# Autodesk Inventor assembly: Gear
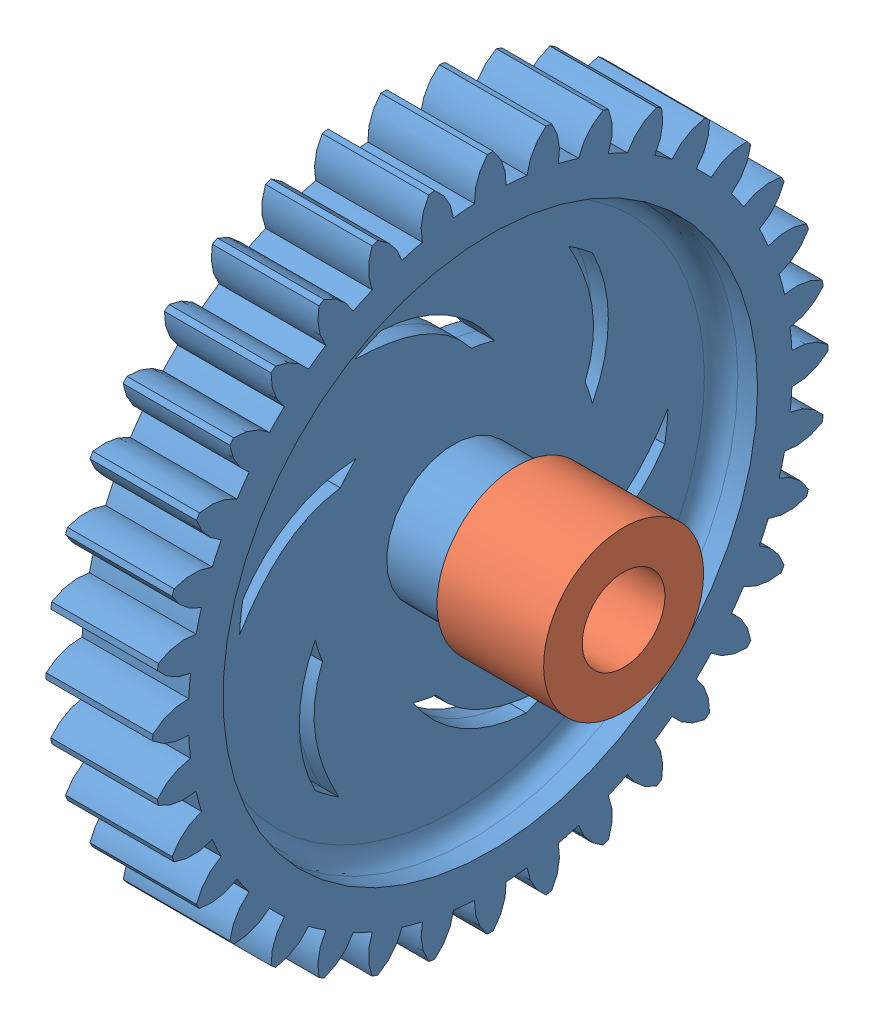
[picture p0: shaded view drawn from the shape stored in the file]
Saved by Autodesk Inventor 2025 (Build 290162000, 162)
## iProperties
Created: 2025-01-28
Part Number: Gear
Document SubType Name: Assembly
Designer: Averey Ku
Author: Averey Ku
## Documents named in this file (4)
- D:\VEX\High Stakes\CAD\V5\Chassis\Drivebay\Gear.iam
- D:\VEX\High Stakes\CAD\ROBOPROS-CAD-Inventor\Motion\Gears\LS 36T Gear.ipt
- D:\VEX\High Stakes\CAD\ROBOPROS-CAD-Inventor\Motion\Spacers\Spacer Nylon .375 OD\NSpacer .375 OD x .250.ipt
- D:\VEX\High Stakes\CAD\ROBOPROS-CAD-Inventor\Motion\Spacers\Spacer Nylon .375 OD.ipt
## Components (2 placed, 2 different names)
1. LS 36T Gear:1 — Insert:1
2. NSpacer .375 OD x .250:1 — Insert:1
## Relationships (1: Insert 1)
- Insert:1: LS 36T Gear:1 ↔ NSpacer .375 OD x .250:1
